# Autodesk Inventor assembly: E-AXIS ASSEMBLY P1.3
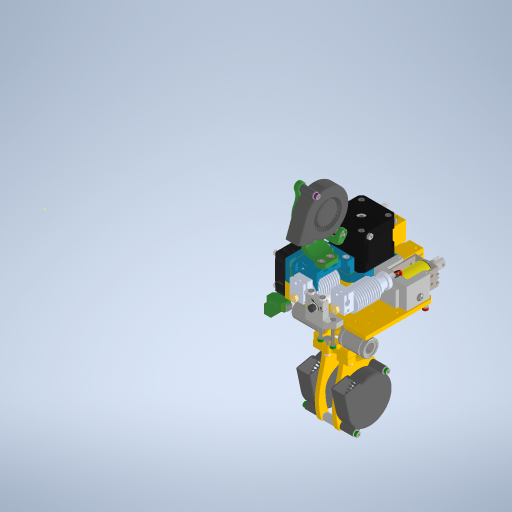
[picture p0: Inventor's stored thumbnail of the model, 512x512]
Saved by Autodesk Inventor 2023 (Build 270158000, 158)
## iProperties
Created: 2019-12-18
Part Number: E-AXIS ASSEMBLY P1.3
Document SubType Name: Assembly
Designer: pepd9
Mass: 917.379 g
Surface Area: 2479.59 cm^2
Volume: 339.663 cm^3
Density: 2.70085 g/cm^3
Author: pepd9
## Documents named in this file (42)
- D:\000 - PEPCORP CLOUD\00- Legacy\Designs\MK3PRO P1\E-Axis\E-AXIS ASSEMBLY P1.3.iam
- D:\000 - PEPCORP CLOUD\00- Legacy\Designs\MK3PRO P1\E-Axis\X-Carriage V1.3.ipt
- D:\000 - PEPCORP CLOUD\00- Legacy\Designs\MK3PRO P1\COMPONENTS\M3 Nut.ipt
- D:\000 - PEPCORP CLOUD\00- Legacy\Designs\MK3PRO P1\COMPONENTS\NUT_SQUARE_M3.ipt
- D:\000 - PEPCORP CLOUD\00- Legacy\Designs\MK3PRO P1\COMPONENTS\LM10UU.ipt
- D:\000 - PEPCORP CLOUD\00- Legacy\Designs\MK3PRO P1\COMPONENTS\SHCS_M3_14.ipt
- D:\000 - PEPCORP CLOUD\00- Legacy\Designs\MK3PRO P1\E-Axis\Endstop Trigger Block.ipt
- D:\000 - PEPCORP CLOUD\00- Legacy\Designs\MK3PRO P1\COMPONENTS\SHCS_M3_20.ipt
- D:\000 - PEPCORP CLOUD\00- Legacy\Designs\MK3PRO P1\E-Axis\Extruder Back V2.ipt
- D:\000 - PEPCORP CLOUD\00- Legacy\Designs\MK3PRO P1\COMPONENTS\SHCS_M3_12.ipt
- D:\000 - PEPCORP CLOUD\00- Legacy\Designs\MK3PRO P1\E-Axis\extruder-cover.ipt
- D:\000 - PEPCORP CLOUD\00- Legacy\Designs\MK3PRO P1\E-Axis\Fan Support Front.ipt
- D:\000 - PEPCORP CLOUD\00- Legacy\Designs\MK3PRO P1\E-Axis\Left Cable Guide.ipt
- D:\000 - PEPCORP CLOUD\00- Legacy\Designs\MK3PRO P1\COMPONENTS\SHCS_M3_35.ipt
- D:\000 - PEPCORP CLOUD\00- Legacy\Designs\MK3PRO P1\COMPONENTS\SHCS_M3_40.ipt
- D:\000 - PEPCORP CLOUD\00- Legacy\Designs\MK3PRO P1\COMPONENTS\Bondtech Idler.ipt
- D:\000 - PEPCORP CLOUD\00- Legacy\Designs\MK3PRO P1\E-Axis\PINDA_Probe.ipt
- D:\000 - PEPCORP CLOUD\00- Legacy\Designs\MK3PRO P1\E-Axis\E3D_V6.ipt
- D:\000 - PEPCORP CLOUD\00- Legacy\Designs\MK3PRO P1\E-Axis\E-Motor Mount P1.1.ipt
- D:\000 - PEPCORP CLOUD\00- Legacy\Designs\MK3PRO P1\E-Axis\Extruder_stepper_motor.iam
- D:\000 - PEPCORP CLOUD\00- Legacy\Designs\MK3PRO P1\COMPONENTS\SHCS_M3_8.ipt
- D:\000 - PEPCORP CLOUD\00- Legacy\Designs\MK3PRO P1\COMPONENTS\Bondtech Driver.ipt
- D:\000 - PEPCORP CLOUD\00- Legacy\Designs\MK3PRO P1\COMPONENTS\M3 Washer.ipt
- D:\000 - PEPCORP CLOUD\00- Legacy\Designs\MK3PRO P1\COMPONENTS\SHCS_M3_30.ipt
- D:\000 - PEPCORP CLOUD\00- Legacy\Designs\MK3PRO P1\COMPONENTS\FAN_5015_BLOWER.ipt
- D:\000 - PEPCORP CLOUD\00- Legacy\Designs\MK3PRO P1\COMPONENTS\SHCS_M3_25.ipt
- D:\000 - PEPCORP CLOUD\00- Legacy\Designs\MK3PRO P1\E-Axis\x-Carriage Backplate V1.2.ipt
- D:\000 - PEPCORP CLOUD\00- Legacy\Designs\MK3PRO P1\COMPONENTS\SHCS_M3_18.ipt
- D:\000 - PEPCORP CLOUD\00- Legacy\Designs\MK3PRO P1\E-Axis\LimitSwitch Container.ipt
- D:\000 - PEPCORP CLOUD\00- Legacy\Designs\MK3PRO P1\COMPONENTS\Noctua-NF-A4x10.ipt
- D:\000 - PEPCORP CLOUD\00- Legacy\Designs\MK3PRO P1\E-Axis\S Fan Cover.ipt
- D:\000 - PEPCORP CLOUD\00- Legacy\Designs\MK3PRO P1\COMPONENTS\Small Limit Switch.iam
- D:\000 - PEPCORP CLOUD\00- Legacy\Designs\MK3PRO P1\E-Axis\Extruder Cable Clamp.ipt
- D:\000 - PEPCORP CLOUD\00- Legacy\Designs\MK3PRO P1\E-Axis\Rear Fan Backplate Mount.ipt
- D:\000 - PEPCORP CLOUD\00- Legacy\Designs\MK3PRO P1\E-Axis\Rear Left Fan Mount.ipt
- D:\000 - PEPCORP CLOUD\00- Legacy\Designs\MK3PRO P1\E-Axis\Rear Right Fan Mount.ipt
- D:\000 - PEPCORP CLOUD\00- Legacy\Designs\MK3PRO P1\E-Axis\Rear Fan Spacer.ipt
- D:\000 - PEPCORP CLOUD\00- Legacy\Designs\MK3PRO P1\E2\Solenoid Assembly.iam
- D:\000 - PEPCORP CLOUD\00- Legacy\Designs\MK3PRO P1\E2\SolenoidBracket.ipt
- D:\000 - PEPCORP CLOUD\00- Legacy\Designs\MK3PRO P1\E-Axis\Extruder Idler V3.ipt
- D:\000 - PEPCORP CLOUD\00- Legacy\Designs\MK3PRO P1\PindaHolder.ipt
- D:\000 - PEPCORP CLOUD\00- Legacy\Designs\MK3PRO P1\COMPONENTS\BHCS M4x8.ipt
## Components (123 placed, 41 different names)
1. X-Carriage V1.3:1 — Flush:1, Mate:1, Mate:2, Mate:3, Mate:4, Mate:5, Mate:6, Mate:7, Mate:8, Mate:9, Mate:14, Mate:15, Mate:16, Mate:17, Mate:18, Mate:19, Mate:20, Angle:1, Angle:2, Angle:3, Angle:4, Angle:5, Angle:6, Angle:7, Mate:21, Mate:22, Angle:10, Mate:23, Mate:24, Mate:25, Mate:26, Mate:27, Mate:28, Mate:29, Mate:30, Mate:31, Mate:32, Mate:33, Mate:34, Angle:11, Mate:35, Mate:36, Angle:12, Mate:49, Mate:50, Mate:51, Mate:58, Mate:59, Mate:60, Mate:61, Mate:68, Mate:69, Mate:70, Mate:71, Mate:72, Mate:73, Mate:145, Mate:146, Mate:147, Mate:404, Mate:405, Mate:406, Mate:407
2. M3 Nut:1 — Mate:6, Mate:15, Angle:6
3. M3 Nut:2 — Mate:7, Mate:16, Angle:5
4. M3 Nut:3 — Mate:9, Mate:18, Angle:3
5. M3 Nut:4 — Mate:8, Mate:17, Angle:4
6. M3 Nut:5 — Mate:4, Mate:19, Angle:2
7. M3 Nut:6 — Mate:3, Mate:20, Angle:1
8. M3 Nut:7 — Mate:5, Mate:14, Angle:7
9. NUT_SQUARE_M3:1 — Mate:21, Mate:22, Angle:10
10. LM10UU:1 — Mate:25, Mate:28
11. LM10UU:2 — Mate:24, Mate:27
12. LM10UU:3 — Mate:23, Mate:26
13. SHCS_M3_14:1 — Mate:30, Mate:32
14. SHCS_M3_14:2 — Mate:29, Mate:31
15. Endstop Trigger Block:1 — Mate:35, Mate:36, Angle:12, Mate:37, Mate:38
16. NUT_SQUARE_M3:2 — Mate:33, Mate:34, Angle:11
17. SHCS_M3_20:1 — Mate:37, Mate:38
18. Extruder Back V2:1 — Mate:39, Mate:40, Mate:41, Mate:42, Mate:43, Mate:44, Mate:45, Mate:46, Angle:13, Mate:47, Angle:14, Mate:48, Angle:15, Mate:49, Mate:50, Mate:51, Mate:52, Mate:53, Angle:16, Mate:54, Mate:55, Mate:56, Mate:57, Angle:17, Angle:18, Mate:62, Mate:63, Angle:19, Mate:76, Mate:77, Mate:80, Mate:81, Angle:21, Mate:88, Mate:89, Mate:90, Mate:164, Mate:165, Angle:35, Mate:168, Mate:169, Mate:170, Angle:54, Mate:281, Mate:282, Mate:379, Flush:17
19. M3 Nut:10 — Mate:39, Mate:41
20. M3 Nut:11 — Mate:40, Mate:42
21. NUT_SQUARE_M3:3 — Mate:45, Mate:46, Angle:13
22. NUT_SQUARE_M3:4 — Mate:44, Mate:47, Angle:14
23. NUT_SQUARE_M3:5 — Mate:43, Mate:48, Angle:15
24. NUT_SQUARE_M3:6 — Mate:52, Mate:53, Angle:16
25. M3 Nut:12 — Mate:54, Mate:57, Angle:18
26. M3 Nut:13 — Mate:55, Mate:56, Angle:17
27. SHCS_M3_12:1 — Mate:58, Mate:60
28. SHCS_M3_12:2 — Mate:59, Mate:61
29. extruder-cover:1 — Mate:96, Mate:97, Mate:98, Mate:99, Mate:100, Mate:101, Angle:24, Mate:102, Angle:25, Mate:103, Mate:104, Angle:26, Mate:105, Mate:106, Angle:27, Mate:107, Mate:108, Mate:109, Mate:110, Mate:111, Mate:112, Mate:113
30. Fan Support Front:1 — Mate:111, Mate:112, Mate:113, Mate:114, Mate:115, Mate:116, Mate:117, Mate:118, Mate:119, Angle:28, Mate:120, Mate:121, Angle:29, Mate:124, Mate:125, Mate:126, Mate:131, Mate:132
31. Left Cable Guide:1 — Mate:62, Mate:63, Angle:19, Mate:64, Mate:65, Angle:20, Mate:66, Mate:67, Mate:266, Mate:267, Angle:53, Mate:268, Mate:269, Mate:270
32. NUT_SQUARE_M3:7 — Mate:64, Mate:65, Angle:20
33. SHCS_M3_12:3 — Mate:66, Mate:67
34. SHCS_M3_35:1 — Mate:68, Mate:71
35. SHCS_M3_35:2 — Mate:70, Mate:73
36. SHCS_M3_35:3 — Mate:69, Mate:72
37. SHCS_M3_40:1 — Mate:76, Mate:77, Mate:94, Mate:95, Mate:384
38. Bondtech Idler:1 — Flush:3, Mate:380
39. PINDA_Probe:1 — Flush:2, Mate:408, Flush:18
40. E3D_V6:1 — Mate:80, Mate:81, Angle:21, Flush:2, Angle:63, Flush:18
41. E-Motor Mount P1.1:1 — Mate:83, Mate:84, Mate:85, Mate:86, Mate:87, Mate:88, Mate:89, Mate:90, Mate:96, Mate:97, Mate:98, Mate:380, Mate:381, Mate:382, Angle:67
42. Extruder_stepper_motor:1 [sub-assembly] — Mate:83, Mate:84, Mate:85, Mate:91
43. SHCS_M3_8:1 — Mate:86, Mate:87
44. Bondtech Driver:1 — Mate:91, Flush:3
45. M3 Washer:1 — Mate:383, Mate:384
46. M3 Washer:2 — Mate:94, Mate:95
47. NUT_SQUARE_M3:8 — Mate:105, Mate:106, Angle:27
48. NUT_SQUARE_M3:9 — Mate:103, Mate:104, Angle:26
49. NUT_SQUARE_M3:10 — Mate:100, Mate:101, Angle:24
50. NUT_SQUARE_M3:11 — Mate:99, Mate:102, Angle:25
51. SHCS_M3_30:1 — Mate:107, Mate:108
52. SHCS_M3_30:2 — Mate:109, Mate:110
53. M3 Nut:14 — Mate:118, Mate:119, Angle:28
54. M3 Nut:15 — Mate:120, Mate:121, Angle:29
55. SHCS_M3_8:2 — Mate:114, Mate:117
56. SHCS_M3_8:3 — Mate:115, Mate:116
57. FAN_5015_BLOWER:1 — Mate:124, Mate:125, Mate:126, Mate:127, Mate:128
58. SHCS_M3_20:2 — Mate:127, Mate:129, Mate:130
59. M3 Washer:3 — Mate:128, Mate:129, Mate:130
60. SHCS_M3_25:1 — Mate:131, Mate:132
61. x-Carriage Backplate V1.2:1 — Mate:141, Mate:142, Mate:143, Mate:144, Angle:33, Angle:34, Mate:145, Mate:146, Mate:147, Mate:148, Mate:149, Mate:150, Mate:151, Mate:152, Mate:153, Mate:154, Mate:155, Mate:160, Mate:161, Mate:162, Mate:163, Mate:187, Mate:214, Mate:275, Mate:387, Mate:388, Mate:389, Mate:390
62. M3 Nut:18 — Mate:141, Mate:144, Angle:33
63. M3 Nut:19 — Mate:142, Mate:143, Angle:34
64. SHCS_M3_18:1 — Mate:148, Mate:153
65. SHCS_M3_18:2 — Mate:149, Mate:151
66. SHCS_M3_18:3 — Mate:150, Mate:152
67. SHCS_M3_18:4 — Mate:154, Mate:155
68. SHCS_M3_18:7 — Mate:160, Mate:163
69. SHCS_M3_18:8 — Mate:161, Mate:162
70. LimitSwitch Container:1 — Mate:164, Mate:165, Angle:35, Mate:166, Mate:167, Mate:179, Mate:180, Mate:181
71. SHCS_M3_8:4 — Mate:166, Mate:167
72. Noctua-NF-A4x10:1 — Mate:168, Mate:169, Mate:170, Mate:171, Mate:172, Mate:173, Mate:174, Mate:248
73. SHCS_M3_18:9 — Mate:172, Mate:249
74. SHCS_M3_18:10 — Mate:171
75. SHCS_M3_18:11 — Mate:173, Mate:250
76. SHCS_M3_18:12 — Mate:174
77. Small Limit Switch:1 [sub-assembly] — Mate:179, Mate:180, Mate:181
78. Rear Fan Backplate Mount:1 — Mate:182, Mate:183, Mate:184, Mate:185, Angle:37, Mate:187, Mate:188, Mate:189, Mate:190, Mate:191, Mate:200, Mate:201, Mate:202, Mate:203, Angle:52, Mate:275
79. M3 Nut:20 — Mate:182, Mate:184
80. M3 Nut:21 — Mate:183, Mate:185, Angle:37
81. SHCS_M3_12:6 — Mate:188, Mate:189
82. SHCS_M3_14:3 — Mate:190, Mate:191, Mate:214
83. Rear Left Fan Mount:1 — Mate:198, Angle:40, Mate:201, Mate:202, Mate:205, Mate:206, Mate:207, Mate:219, Mate:222, Angle:52, Mate:374, Angle:66
84. Rear Right Fan Mount:1 — Mate:196, Angle:42, Mate:200, Mate:203, Mate:204, Mate:208, Mate:209, Mate:220, Mate:221, Mate:373, Angle:65, Mate:377
85. M3 Nut:22 — Mate:196, Angle:42, Mate:265
86. M3 Nut:25 — Mate:198, Angle:40, Mate:246
87. FAN_5015_BLOWER:2 — Mate:204, Mate:208, Mate:209, Mate:242, Mate:243, Mate:255, Mate:256
88. FAN_5015_BLOWER:3 — Mate:205, Mate:206, Mate:207, Mate:240, Mate:241, Mate:371, Mate:372
89. SHCS_M3_14:4 — Mate:219, Mate:222
90. SHCS_M3_14:5 — Mate:220, Mate:221
91. SHCS_M3_25:2 — Mate:240, Mate:241, Mate:247
92. SHCS_M3_25:3 — Mate:242, Mate:244, Mate:245
93. M3 Washer:4 — Mate:243, Mate:244, Mate:245
94. Rear Fan Spacer:1 — Mate:246, Mate:247, Mate:265
95. S Fan Cover:1 — Mate:248, Mate:249, Mate:250
96. SHCS_M3_18:13 — Mate:271, Mate:274
97. SHCS_M3_25:4 — Mate:255, Mate:257, Mate:258, Mate:376, Mate:378
98. M3 Washer:5 — Mate:256, Mate:257, Mate:258
99. NUT_SQUARE_M3:12 — Mate:266, Mate:267, Angle:53
100. SHCS_M3_18:14 — Mate:272, Mate:273
101. Extruder Cable Clamp:1 — Mate:268, Mate:269, Mate:270, Mate:271, Mate:272, Mate:273, Mate:274
102. Solenoid Assembly:1 [sub-assembly] — Angle:54, Mate:278, Mate:403, Angle:70
103. SolenoidBracket:1 — Mate:278, Mate:281, Mate:282, Mate:403, Angle:70, Mate:444, Mate:445, Mate:446, Mate:447
104. E3D_V6:2 — Angle:63
105. SHCS_M3_25:5 — Mate:371, Mate:372, Mate:375
106. M3 Nut:26 — Mate:373, Mate:376, Angle:65
107. M3 Nut:27 — Mate:374, Mate:375, Angle:66
108. Rear Fan Spacer:2 — Mate:377, Mate:378
109. Extruder Idler V3:1 — Mate:381, Mate:382, Angle:67, Mate:383
110. PindaHolder:1 — Flush:17, Mate:391, Mate:392, Angle:68, Mate:393, Angle:69, Mate:395, Mate:396, Mate:397, Mate:398, Mate:399, Mate:400, Mate:401, Mate:402, Mate:408
111. SHCS_M3_25:6 — Mate:387, Mate:390
112. SHCS_M3_25:7 — Mate:388, Mate:389, Mate:394
113. M3 Nut:28 — Mate:391, Mate:392, Angle:68
114. M3 Nut:29 — Mate:393, Mate:394, Angle:69
115. NUT_SQUARE_M3:13 — Mate:395, Mate:396
116. NUT_SQUARE_M3:14 — Mate:397, Mate:398
117. SHCS_M3_18:15 — Mate:399, Mate:401
118. SHCS_M3_18:16 — Mate:400, Mate:402
119. SHCS_M3_35:4 — Mate:404, Mate:407
120. SHCS_M3_35:5 — Mate:405, Mate:406
121. M3 Nut:30
122. BHCS M4x8:1 — Mate:446, Mate:447
123. BHCS M4x8:2 — Mate:444, Mate:445
## Relationships (293: Mate 247, Angle 41, Flush 5)
- Flush:1: X-Carriage V1.3:1
- Mate:1 (8.3 mm): X-Carriage V1.3:1
- Mate:2 (-43.75 mm): X-Carriage V1.3:1
- Mate:3: X-Carriage V1.3:1 ↔ M3 Nut:6
- Mate:4: X-Carriage V1.3:1 ↔ M3 Nut:5
- Mate:5: X-Carriage V1.3:1 ↔ M3 Nut:7
- Mate:6: X-Carriage V1.3:1 ↔ M3 Nut:1
- Mate:7: X-Carriage V1.3:1 ↔ M3 Nut:2
- Mate:8: X-Carriage V1.3:1 ↔ M3 Nut:4
- Mate:9: X-Carriage V1.3:1 ↔ M3 Nut:3
- Mate:14: X-Carriage V1.3:1 ↔ M3 Nut:7
- Mate:15: X-Carriage V1.3:1 ↔ M3 Nut:1
- Mate:16: X-Carriage V1.3:1 ↔ M3 Nut:2
- Mate:17: X-Carriage V1.3:1 ↔ M3 Nut:4
- Mate:18: X-Carriage V1.3:1 ↔ M3 Nut:3
- Mate:19: X-Carriage V1.3:1 ↔ M3 Nut:5
- Mate:20: X-Carriage V1.3:1 ↔ M3 Nut:6
- Angle:1 (0 deg): X-Carriage V1.3:1 ↔ M3 Nut:6
- Angle:2 (0 deg): X-Carriage V1.3:1 ↔ M3 Nut:5
- Angle:3 (0 deg): X-Carriage V1.3:1 ↔ M3 Nut:3
- Angle:4 (0 deg): X-Carriage V1.3:1 ↔ M3 Nut:4
- Angle:5 (0 deg): X-Carriage V1.3:1 ↔ M3 Nut:2
- Angle:6 (0 deg): X-Carriage V1.3:1 ↔ M3 Nut:1
- Angle:7 (0 deg): X-Carriage V1.3:1 ↔ M3 Nut:7
- Mate:21: X-Carriage V1.3:1 ↔ NUT_SQUARE_M3:1
- Mate:22: X-Carriage V1.3:1 ↔ NUT_SQUARE_M3:1
- Angle:10 (0 deg): X-Carriage V1.3:1 ↔ NUT_SQUARE_M3:1
- Mate:23: X-Carriage V1.3:1 ↔ LM10UU:3
- Mate:24: X-Carriage V1.3:1 ↔ LM10UU:2
- Mate:25: X-Carriage V1.3:1 ↔ LM10UU:1
- Mate:26 (0.25 mm): X-Carriage V1.3:1 ↔ LM10UU:3
- Mate:27 (0.25 mm): X-Carriage V1.3:1 ↔ LM10UU:2
- Mate:28 (0.25 mm): X-Carriage V1.3:1 ↔ LM10UU:1
- Mate:29: X-Carriage V1.3:1 ↔ SHCS_M3_14:2
- Mate:30: X-Carriage V1.3:1 ↔ SHCS_M3_14:1
- Mate:31: X-Carriage V1.3:1 ↔ SHCS_M3_14:2
- Mate:32: X-Carriage V1.3:1 ↔ SHCS_M3_14:1
- Mate:33: X-Carriage V1.3:1 ↔ NUT_SQUARE_M3:2
- Mate:34: X-Carriage V1.3:1 ↔ NUT_SQUARE_M3:2
- Angle:11 (0 deg): X-Carriage V1.3:1 ↔ NUT_SQUARE_M3:2
- Mate:35: X-Carriage V1.3:1 ↔ Endstop Trigger Block:1
- Mate:36: X-Carriage V1.3:1 ↔ Endstop Trigger Block:1
- Angle:12 (180 deg): X-Carriage V1.3:1 ↔ Endstop Trigger Block:1
- Mate:37: Endstop Trigger Block:1 ↔ SHCS_M3_20:1
- Mate:38: Endstop Trigger Block:1 ↔ SHCS_M3_20:1
- Mate:39: Extruder Back V2:1 ↔ M3 Nut:10
- Mate:40: Extruder Back V2:1 ↔ M3 Nut:11
- Mate:41: Extruder Back V2:1 ↔ M3 Nut:10
- Mate:42: Extruder Back V2:1 ↔ M3 Nut:11
- Mate:43: Extruder Back V2:1 ↔ NUT_SQUARE_M3:5
- Mate:44: Extruder Back V2:1 ↔ NUT_SQUARE_M3:4
- Mate:45: Extruder Back V2:1 ↔ NUT_SQUARE_M3:3
- Mate:46: Extruder Back V2:1 ↔ NUT_SQUARE_M3:3
- Angle:13 (0 deg): Extruder Back V2:1 ↔ NUT_SQUARE_M3:3
- Mate:47: Extruder Back V2:1 ↔ NUT_SQUARE_M3:4
- Angle:14 (0 deg): Extruder Back V2:1 ↔ NUT_SQUARE_M3:4
- Mate:48: Extruder Back V2:1 ↔ NUT_SQUARE_M3:5
- Angle:15 (0 deg): Extruder Back V2:1 ↔ NUT_SQUARE_M3:5
- Mate:49: X-Carriage V1.3:1 ↔ Extruder Back V2:1
- Mate:50: X-Carriage V1.3:1 ↔ Extruder Back V2:1
- Mate:51: X-Carriage V1.3:1 ↔ Extruder Back V2:1
- Mate:52: Extruder Back V2:1 ↔ NUT_SQUARE_M3:6
- Mate:53: Extruder Back V2:1 ↔ NUT_SQUARE_M3:6
- Angle:16 (0 deg): Extruder Back V2:1 ↔ NUT_SQUARE_M3:6
- Mate:54: Extruder Back V2:1 ↔ M3 Nut:12
- Mate:55: Extruder Back V2:1 ↔ M3 Nut:13
- Mate:56: Extruder Back V2:1 ↔ M3 Nut:13
- Mate:57: Extruder Back V2:1 ↔ M3 Nut:12
- Angle:17 (0 deg): Extruder Back V2:1 ↔ M3 Nut:13
- Angle:18 (0 deg): Extruder Back V2:1 ↔ M3 Nut:12
- Mate:58: X-Carriage V1.3:1 ↔ SHCS_M3_12:1
- Mate:59: X-Carriage V1.3:1 ↔ SHCS_M3_12:2
- Mate:60: X-Carriage V1.3:1 ↔ SHCS_M3_12:1
- Mate:61: X-Carriage V1.3:1 ↔ SHCS_M3_12:2
- Mate:62: Extruder Back V2:1 ↔ Left Cable Guide:1
- Mate:63: Extruder Back V2:1 ↔ Left Cable Guide:1
- Angle:19 (180 deg): Extruder Back V2:1 ↔ Left Cable Guide:1
- Mate:64: Left Cable Guide:1 ↔ NUT_SQUARE_M3:7
- Mate:65: Left Cable Guide:1 ↔ NUT_SQUARE_M3:7
- Angle:20 (0 deg): Left Cable Guide:1 ↔ NUT_SQUARE_M3:7
- Mate:66: Left Cable Guide:1 ↔ SHCS_M3_12:3
- Mate:67: Left Cable Guide:1 ↔ SHCS_M3_12:3
- Mate:68: X-Carriage V1.3:1 ↔ SHCS_M3_35:1
- Mate:69: X-Carriage V1.3:1 ↔ SHCS_M3_35:3
- Mate:70: X-Carriage V1.3:1 ↔ SHCS_M3_35:2
- Mate:71: X-Carriage V1.3:1 ↔ SHCS_M3_35:1
- Mate:72: X-Carriage V1.3:1 ↔ SHCS_M3_35:3
- Mate:73: X-Carriage V1.3:1 ↔ SHCS_M3_35:2
- Mate:76: Extruder Back V2:1 ↔ SHCS_M3_40:1
- Mate:77: Extruder Back V2:1 ↔ SHCS_M3_40:1
- Mate:80: Extruder Back V2:1 ↔ E3D_V6:1
- Mate:81: Extruder Back V2:1 ↔ E3D_V6:1
- Angle:21 (90 deg): Extruder Back V2:1 ↔ E3D_V6:1
- Flush:2 (2 mm): PINDA_Probe:1 ↔ E3D_V6:1
- Mate:83: E-Motor Mount P1.1:1 ↔ Extruder_stepper_motor:1
- Mate:84: E-Motor Mount P1.1:1 ↔ Extruder_stepper_motor:1
- Mate:85: E-Motor Mount P1.1:1 ↔ Extruder_stepper_motor:1
- Mate:86: E-Motor Mount P1.1:1 ↔ SHCS_M3_8:1
- Mate:87: E-Motor Mount P1.1:1 ↔ SHCS_M3_8:1
- Mate:88: Extruder Back V2:1 ↔ E-Motor Mount P1.1:1
- Mate:89: Extruder Back V2:1 ↔ E-Motor Mount P1.1:1
- Mate:90: Extruder Back V2:1 ↔ E-Motor Mount P1.1:1
- Mate:91: Extruder_stepper_motor:1 ↔ Bondtech Driver:1
- Flush:3: Bondtech Idler:1 ↔ Bondtech Driver:1
- Mate:94: SHCS_M3_40:1 ↔ M3 Washer:2
- Mate:95: SHCS_M3_40:1 ↔ M3 Washer:2
- Mate:96: extruder-cover:1 ↔ E-Motor Mount P1.1:1
- Mate:97: extruder-cover:1 ↔ E-Motor Mount P1.1:1
- Mate:98: extruder-cover:1 ↔ E-Motor Mount P1.1:1
- Mate:99: extruder-cover:1 ↔ NUT_SQUARE_M3:11
- Mate:100: extruder-cover:1 ↔ NUT_SQUARE_M3:10
- Mate:101: extruder-cover:1 ↔ NUT_SQUARE_M3:10
- Angle:24 (0 deg): extruder-cover:1 ↔ NUT_SQUARE_M3:10
- Mate:102: extruder-cover:1 ↔ NUT_SQUARE_M3:11
- Angle:25 (0 deg): extruder-cover:1 ↔ NUT_SQUARE_M3:11
- Mate:103: extruder-cover:1 ↔ NUT_SQUARE_M3:9
- Mate:104: extruder-cover:1 ↔ NUT_SQUARE_M3:9
- Angle:26 (0 deg): extruder-cover:1 ↔ NUT_SQUARE_M3:9
- Mate:105: extruder-cover:1 ↔ NUT_SQUARE_M3:8
- Mate:106: extruder-cover:1 ↔ NUT_SQUARE_M3:8
- Angle:27 (0 deg): extruder-cover:1 ↔ NUT_SQUARE_M3:8
- Mate:107: extruder-cover:1 ↔ SHCS_M3_30:1
- Mate:108: extruder-cover:1 ↔ SHCS_M3_30:1
- Mate:109: extruder-cover:1 ↔ SHCS_M3_30:2
- Mate:110: extruder-cover:1 ↔ SHCS_M3_30:2
- Mate:111: extruder-cover:1 ↔ Fan Support Front:1
- Mate:112: extruder-cover:1 ↔ Fan Support Front:1
- Mate:113: extruder-cover:1 ↔ Fan Support Front:1
- Mate:114: Fan Support Front:1 ↔ SHCS_M3_8:2
- Mate:115: Fan Support Front:1 ↔ SHCS_M3_8:3
- Mate:116: Fan Support Front:1 ↔ SHCS_M3_8:3
- Mate:117: Fan Support Front:1 ↔ SHCS_M3_8:2
- Mate:118: Fan Support Front:1 ↔ M3 Nut:14
- Mate:119: Fan Support Front:1 ↔ M3 Nut:14
- Angle:28 (0 deg): Fan Support Front:1 ↔ M3 Nut:14
- Mate:120: Fan Support Front:1 ↔ M3 Nut:15
- Mate:121: Fan Support Front:1 ↔ M3 Nut:15
- Angle:29 (30 deg): Fan Support Front:1 ↔ M3 Nut:15
- Mate:124: Fan Support Front:1 ↔ FAN_5015_BLOWER:1
- Mate:125: Fan Support Front:1 ↔ FAN_5015_BLOWER:1
- Mate:126: Fan Support Front:1 ↔ FAN_5015_BLOWER:1
- Mate:127: FAN_5015_BLOWER:1 ↔ SHCS_M3_20:2
- Mate:128: FAN_5015_BLOWER:1 ↔ M3 Washer:3
- Mate:129: SHCS_M3_20:2 ↔ M3 Washer:3
- Mate:130: SHCS_M3_20:2 ↔ M3 Washer:3
- Mate:131: Fan Support Front:1 ↔ SHCS_M3_25:1
- Mate:132: Fan Support Front:1 ↔ SHCS_M3_25:1
- Mate:141: x-Carriage Backplate V1.2:1 ↔ M3 Nut:18
- Mate:142: x-Carriage Backplate V1.2:1 ↔ M3 Nut:19
- Mate:143: x-Carriage Backplate V1.2:1 ↔ M3 Nut:19
- Mate:144: x-Carriage Backplate V1.2:1 ↔ M3 Nut:18
- Angle:33 (0 deg): x-Carriage Backplate V1.2:1 ↔ M3 Nut:18
- Angle:34 (0 deg): x-Carriage Backplate V1.2:1 ↔ M3 Nut:19
- Mate:145: X-Carriage V1.3:1 ↔ x-Carriage Backplate V1.2:1
- Mate:146: X-Carriage V1.3:1 ↔ x-Carriage Backplate V1.2:1
- Mate:147: X-Carriage V1.3:1 ↔ x-Carriage Backplate V1.2:1
- Mate:148: x-Carriage Backplate V1.2:1 ↔ SHCS_M3_18:1
- Mate:149: x-Carriage Backplate V1.2:1 ↔ SHCS_M3_18:2
- Mate:150: x-Carriage Backplate V1.2:1 ↔ SHCS_M3_18:3
- Mate:151: x-Carriage Backplate V1.2:1 ↔ SHCS_M3_18:2
- Mate:152: x-Carriage Backplate V1.2:1 ↔ SHCS_M3_18:3
- Mate:153: x-Carriage Backplate V1.2:1 ↔ SHCS_M3_18:1
- Mate:154: x-Carriage Backplate V1.2:1 ↔ SHCS_M3_18:4
- Mate:155: x-Carriage Backplate V1.2:1 ↔ SHCS_M3_18:4
- Mate:160: x-Carriage Backplate V1.2:1 ↔ SHCS_M3_18:7
- Mate:161: x-Carriage Backplate V1.2:1 ↔ SHCS_M3_18:8
- Mate:162: x-Carriage Backplate V1.2:1 ↔ SHCS_M3_18:8
- Mate:163: x-Carriage Backplate V1.2:1 ↔ SHCS_M3_18:7
- Mate:164: Extruder Back V2:1 ↔ LimitSwitch Container:1
- Mate:165: Extruder Back V2:1 ↔ LimitSwitch Container:1
- Angle:35 (180 deg): Extruder Back V2:1 ↔ LimitSwitch Container:1
- Mate:166: LimitSwitch Container:1 ↔ SHCS_M3_8:4
- Mate:167: LimitSwitch Container:1 ↔ SHCS_M3_8:4
- Mate:168: Extruder Back V2:1 ↔ Noctua-NF-A4x10:1
- Mate:169: Extruder Back V2:1 ↔ Noctua-NF-A4x10:1
- Mate:170: Extruder Back V2:1 ↔ Noctua-NF-A4x10:1
- Mate:171: Noctua-NF-A4x10:1 ↔ SHCS_M3_18:10
- Mate:172: Noctua-NF-A4x10:1 ↔ SHCS_M3_18:9
- Mate:173: Noctua-NF-A4x10:1 ↔ SHCS_M3_18:11
- Mate:174: Noctua-NF-A4x10:1 ↔ SHCS_M3_18:12
- Mate:179: LimitSwitch Container:1 ↔ Small Limit Switch:1
- Mate:180: LimitSwitch Container:1 ↔ Small Limit Switch:1
- Mate:181: LimitSwitch Container:1 ↔ Small Limit Switch:1
- Mate:182: Rear Fan Backplate Mount:1 ↔ M3 Nut:20
- Mate:183: Rear Fan Backplate Mount:1 ↔ M3 Nut:21
- Mate:184: Rear Fan Backplate Mount:1 ↔ M3 Nut:20
- Mate:185: Rear Fan Backplate Mount:1 ↔ M3 Nut:21
- Angle:37 (0 deg): Rear Fan Backplate Mount:1 ↔ M3 Nut:21
- Mate:187: x-Carriage Backplate V1.2:1 ↔ Rear Fan Backplate Mount:1
- Mate:188: Rear Fan Backplate Mount:1 ↔ SHCS_M3_12:6
- Mate:189: Rear Fan Backplate Mount:1 ↔ SHCS_M3_12:6
- Mate:190: Rear Fan Backplate Mount:1 ↔ SHCS_M3_14:3
- Mate:191: Rear Fan Backplate Mount:1 ↔ SHCS_M3_14:3
- Mate:196: Rear Right Fan Mount:1 ↔ M3 Nut:22
- Mate:198: Rear Left Fan Mount:1 ↔ M3 Nut:25
- Angle:40 (0 deg): Rear Left Fan Mount:1 ↔ M3 Nut:25
- Angle:42 (0 deg): Rear Right Fan Mount:1 ↔ M3 Nut:22
- Mate:200: Rear Fan Backplate Mount:1 ↔ Rear Right Fan Mount:1
- Mate:201: Rear Fan Backplate Mount:1 ↔ Rear Left Fan Mount:1
- Mate:202: Rear Fan Backplate Mount:1 ↔ Rear Left Fan Mount:1
- Mate:203: Rear Fan Backplate Mount:1 ↔ Rear Right Fan Mount:1
- Mate:204: Rear Right Fan Mount:1 ↔ FAN_5015_BLOWER:2
- Mate:205: Rear Left Fan Mount:1 ↔ FAN_5015_BLOWER:3
- Mate:206: Rear Left Fan Mount:1 ↔ FAN_5015_BLOWER:3
- Mate:207: Rear Left Fan Mount:1 ↔ FAN_5015_BLOWER:3
- Mate:208: Rear Right Fan Mount:1 ↔ FAN_5015_BLOWER:2
- Mate:209: Rear Right Fan Mount:1 ↔ FAN_5015_BLOWER:2
- Mate:214: x-Carriage Backplate V1.2:1 ↔ SHCS_M3_14:3
- Mate:219: Rear Left Fan Mount:1 ↔ SHCS_M3_14:4
- Mate:220: Rear Right Fan Mount:1 ↔ SHCS_M3_14:5
- Mate:221: Rear Right Fan Mount:1 ↔ SHCS_M3_14:5
- Mate:222: Rear Left Fan Mount:1 ↔ SHCS_M3_14:4
- Mate:240: FAN_5015_BLOWER:3 ↔ SHCS_M3_25:2
- Mate:241: FAN_5015_BLOWER:3 ↔ SHCS_M3_25:2
- Mate:242: FAN_5015_BLOWER:2 ↔ SHCS_M3_25:3
- Mate:243: FAN_5015_BLOWER:2 ↔ M3 Washer:4
- Mate:244: SHCS_M3_25:3 ↔ M3 Washer:4
- Mate:245: SHCS_M3_25:3 ↔ M3 Washer:4
- Mate:246: M3 Nut:25 ↔ Rear Fan Spacer:1
- Mate:247: SHCS_M3_25:2 ↔ Rear Fan Spacer:1
- Mate:248: Noctua-NF-A4x10:1 ↔ S Fan Cover:1
- Mate:249: SHCS_M3_18:9 ↔ S Fan Cover:1
- Mate:250: SHCS_M3_18:11 ↔ S Fan Cover:1
- Mate:255: FAN_5015_BLOWER:2 ↔ SHCS_M3_25:4
- Mate:256: FAN_5015_BLOWER:2 ↔ M3 Washer:5
- Mate:257: SHCS_M3_25:4 ↔ M3 Washer:5
- Mate:258: SHCS_M3_25:4 ↔ M3 Washer:5
- Mate:265: M3 Nut:22 ↔ Rear Fan Spacer:1
- Angle:52 (0 deg): Rear Fan Backplate Mount:1 ↔ Rear Left Fan Mount:1
- Mate:266: Left Cable Guide:1 ↔ NUT_SQUARE_M3:12
- Mate:267: Left Cable Guide:1 ↔ NUT_SQUARE_M3:12
- Angle:53 (0 deg): Left Cable Guide:1 ↔ NUT_SQUARE_M3:12
- Mate:268: Left Cable Guide:1 ↔ Extruder Cable Clamp:1
- Mate:269: Left Cable Guide:1 ↔ Extruder Cable Clamp:1
- Mate:270: Left Cable Guide:1 ↔ Extruder Cable Clamp:1
- Mate:271: SHCS_M3_18:13 ↔ Extruder Cable Clamp:1
- Mate:272: SHCS_M3_18:14 ↔ Extruder Cable Clamp:1
- Mate:273: SHCS_M3_18:14 ↔ Extruder Cable Clamp:1
- Mate:274: SHCS_M3_18:13 ↔ Extruder Cable Clamp:1
- Mate:275: x-Carriage Backplate V1.2:1 ↔ Rear Fan Backplate Mount:1
- Angle:54 (0 deg): Extruder Back V2:1 ↔ Solenoid Assembly:1
- Mate:278: Solenoid Assembly:1 ↔ SolenoidBracket:1
- Mate:281: Extruder Back V2:1 ↔ SolenoidBracket:1
- Mate:282: Extruder Back V2:1 ↔ SolenoidBracket:1
- Angle:63 (0 deg): E3D_V6:1 ↔ E3D_V6:2
- Mate:371: FAN_5015_BLOWER:3 ↔ SHCS_M3_25:5
- Mate:372: FAN_5015_BLOWER:3 ↔ SHCS_M3_25:5
- Mate:373: Rear Right Fan Mount:1 ↔ M3 Nut:26
- Mate:374: Rear Left Fan Mount:1 ↔ M3 Nut:27
- Mate:375: SHCS_M3_25:5 ↔ M3 Nut:27
- Mate:376: SHCS_M3_25:4 ↔ M3 Nut:26
- Angle:65 (0 deg): Rear Right Fan Mount:1 ↔ M3 Nut:26
- Angle:66 (0 deg): Rear Left Fan Mount:1 ↔ M3 Nut:27
- Mate:377: Rear Right Fan Mount:1 ↔ Rear Fan Spacer:2
- Mate:378: SHCS_M3_25:4 ↔ Rear Fan Spacer:2
- Mate:379: Extruder Back V2:1
- Mate:380 (4.6 mm): Bondtech Idler:1 ↔ E-Motor Mount P1.1:1
- Mate:381: E-Motor Mount P1.1:1 ↔ Extruder Idler V3:1
- Mate:382 (0.1 mm): E-Motor Mount P1.1:1 ↔ Extruder Idler V3:1
- Angle:67 (270 deg): E-Motor Mount P1.1:1 ↔ Extruder Idler V3:1
- Mate:383: M3 Washer:1 ↔ Extruder Idler V3:1
- Mate:384: SHCS_M3_40:1 ↔ M3 Washer:1
- Flush:17: Extruder Back V2:1 ↔ PindaHolder:1
- Mate:387: x-Carriage Backplate V1.2:1 ↔ SHCS_M3_25:6
- Mate:388: x-Carriage Backplate V1.2:1 ↔ SHCS_M3_25:7
- Mate:389: x-Carriage Backplate V1.2:1 ↔ SHCS_M3_25:7
- Mate:390: x-Carriage Backplate V1.2:1 ↔ SHCS_M3_25:6
- Mate:391: PindaHolder:1 ↔ M3 Nut:28
- Mate:392: PindaHolder:1 ↔ M3 Nut:28
- Angle:68 (0 deg): PindaHolder:1 ↔ M3 Nut:28
- Mate:393: PindaHolder:1 ↔ M3 Nut:29
- Mate:394: SHCS_M3_25:7 ↔ M3 Nut:29
- Angle:69 (0 deg): PindaHolder:1 ↔ M3 Nut:29
- Mate:395: PindaHolder:1 ↔ NUT_SQUARE_M3:13
- Mate:396: PindaHolder:1 ↔ NUT_SQUARE_M3:13
- Mate:397: PindaHolder:1 ↔ NUT_SQUARE_M3:14
- Mate:398: PindaHolder:1 ↔ NUT_SQUARE_M3:14
- Mate:399: PindaHolder:1 ↔ SHCS_M3_18:15
- Mate:400: PindaHolder:1 ↔ SHCS_M3_18:16
- Mate:401: PindaHolder:1 ↔ SHCS_M3_18:15
- Mate:402: PindaHolder:1 ↔ SHCS_M3_18:16
- Mate:403: Solenoid Assembly:1 ↔ SolenoidBracket:1
- Angle:70 (180 deg): Solenoid Assembly:1 ↔ SolenoidBracket:1
- Mate:404: X-Carriage V1.3:1 ↔ SHCS_M3_35:4
- Mate:405: X-Carriage V1.3:1 ↔ SHCS_M3_35:5
- Mate:406: X-Carriage V1.3:1 ↔ SHCS_M3_35:5
- Mate:407: X-Carriage V1.3:1 ↔ SHCS_M3_35:4
- Mate:408: PINDA_Probe:1 ↔ PindaHolder:1
- Flush:18 (-2 mm): PINDA_Probe:1 ↔ E3D_V6:1
- Mate:444: SolenoidBracket:1 ↔ BHCS M4x8:2
- Mate:445: SolenoidBracket:1 ↔ BHCS M4x8:2
- Mate:446: SolenoidBracket:1 ↔ BHCS M4x8:1
- Mate:447: SolenoidBracket:1 ↔ BHCS M4x8:1
